# Autodesk Inventor assembly: Clutch Concept
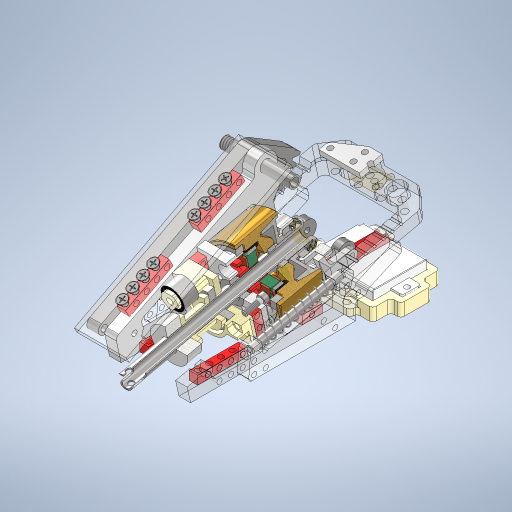
[picture p0: Inventor's stored thumbnail of the model, 512x512]
Saved by Autodesk Inventor 2023.2 (Build 272271000, 271)
## iProperties
Created: 2024-02-03
Part Number: Clutch Concept
Document SubType Name: Assembly
Designer: Nathan Cai
Mass: 1198 g
Surface Area: 3628.58 cm^2
Volume: 470.445 cm^3
Density: 2.54653 g/cm^3
Author: Nathan Cai
## Documents named in this file (50)
- E:\Documents\Inventor\Bleep V1\Clutch Concept.iam
- E:\Documents\Inventor\Bleep V1\Flywheel.ipt
- E:\Documents\Inventor\Bleep V1\Rack.ipt
- E:\Documents\Inventor\Bleep V1\Pin Cap.ipt
- E:\Documents\Inventor\Bleep V1\Thrust Bearing.ipt
- E:\Documents\Inventor\Bleep V1\BB 13x19x4.ipt
- E:\Documents\Inventor\Bleep V1\Cup.ipt
- E:\Documents\Inventor\Bleep V1\1561T741_Stacked Wave Disc Spring\1561T741_Stacked Wave Disc Spring.ipt
- E:\Documents\Inventor\Bleep V1\AKK RS2205 2300KV\AKK RS2205 2300KV.iam
- E:\Documents\Inventor\Bleep V1\Nut Strip 2x1 - 4-40.ipt
- E:\Documents\Inventor\Bleep V1\BB 37mm x 30mm x 4mm.ipt
- E:\Documents\Inventor\Bleep V1\Motor Plate.ipt
- E:\Documents\Inventor\Bleep V1\Uprights.ipt
- E:\Documents\Inventor\Bleep V1\Nut Strip 4x4 - 4-40.ipt
- E:\Documents\Inventor\Bleep V1\5172T23_Metal Gear - 20 Degree Pressure Angle\5172T23_Metal Gear - 20 Degree Pressure Angle.ipt
- E:\Documents\Inventor\Bleep V1\BB .25x.5x.1875 - Flangeless.ipt
- E:\Documents\Inventor\Content Center Files\R2023\en-US\ANSI B18.3(13)\ANSI B18.3 - 4-40 UNC - 0.375(22).ipt
- E:\Documents\Inventor\Bleep V1\Lever.ipt
- E:\Documents\Inventor\Bleep V1\Servo Support.ipt
- E:\Documents\Inventor\Bleep V1\Part1\Part1.ipt
- E:\Documents\Inventor\Bleep V1\Cam - Lever.ipt
- E:\Documents\Inventor\Bleep V1\Cam - Shell.ipt
- E:\Documents\Inventor\Bleep V1\BB 3x7x3.ipt
- E:\Documents\Inventor\Bleep V1\Ramp.ipt
- E:\Documents\Inventor\Content Center Files\R2023\en-US\ANSI B18.6.3(12)\ANSI B18.6.3 - 4-40 UNC - 0.375(15_).ipt
- E:\Documents\Inventor\Content Center Files\R2023\en-US\ISO 4762(2)\ISO 4762 - M3 x 12ISO.ipt
- E:\Documents\Inventor\Content Center Files\R2023\en-US\NF E 25-409\NF E 25-409 - M3.ipt
- E:\Documents\Inventor\Bleep V1\Lever - Copy.ipt
- E:\Documents\Inventor\Bleep V1\Brace.ipt
- E:\Documents\Inventor\Bleep V1\Tattu 4S 850mah\Tattu 850mah 4S.iam
- E:\Documents\Inventor\Bleep V1\BB 3x7x3 - Copy.ipt
- E:\Documents\Inventor\Bleep V1\End Guides - Rail.ipt
- E:\Documents\Inventor\Bleep V1\Spring.ipt
- E:\Documents\Inventor\Bleep V1\Shaft - Arms.ipt
- E:\Documents\Inventor\Bleep V1\Bottom Plate.ipt
- E:\Documents\Inventor\Bleep V1\Side Plate.ipt
- E:\Documents\Inventor\Bleep V1\Top Plate.ipt
- E:\Documents\Inventor\Bleep V1\Back Plate.ipt
- E:\Documents\Inventor\Bleep V1\Uprights- Exterior.ipt
- E:\Documents\Inventor\Bleep V1\Cover.ipt
- E:\Documents\Inventor\Bleep V1\Wheel  - Front.ipt
- E:\Documents\Inventor\Bleep V1\Wheel - Back.ipt
- E:\Documents\Inventor\Bleep V1\Wedge.ipt
- E:\Documents\Inventor\Bleep V1\Ranglebox Mars-25 Assembly - Simple\Ranglebox Mars-25 Assembly - Simple.ipt
- E:\Documents\Inventor\Bleep V1\Shaft - Flywheel C.ipt
- E:\Documents\Inventor\Bleep V1\Clutch C.ipt
- E:\Documents\Inventor\Bleep V1\9293K44_Constant-Force Spring\9293K44_Constant-Force Spring.ipt
- E:\Documents\Inventor\Bleep V1\Spring Mount.ipt
- E:\Documents\Inventor\Bleep V1\Spring Spool.ipt
- E:\Documents\Inventor\Bleep V1\Collar.ipt
## Components (96 placed, 49 different names)
1. 9293K44_Constant-Force Spring:1 — Mate:323, Tangent:2
2. Spring Mount:1 — Mate:316, Flush:149, Mate:317, Mate:320, Mate:323, Tangent:2
3. Thrust Bearing:1 — Mate:319, Mate:320, Mate:322
4. Spring Spool:1 — Mate:321, Mate:322, Mate:325
5. Collar:1 — Mate:324, Mate:325
6. Flywheel:1 — Mate:37, Flush:102, Mate:104, Mate:105, Mate:275, Mate:309
7. Shaft - Flywheel C:1 — Mate:306, Mate:307, Mate:308, Mate:310, Mate:311, Mate:312, Mate:313, Mate:314, Mate:315, Angle:4, Mate:319, Mate:321, Mate:324
8. Shaft - Arms:1 — Mate:257, Flush:118, Mate:288, Mate:291
9. Clutch C:1 — Mate:308, Angle:4
10. Rack:1 — Flush:5, Mate:17, Mate:19, Angle:1, Angle:3, Rotation/Translation:1, Mate:315, Mate:258, Mate:259, Mate:260, Mate:261, Flush:122, Mate:313, Mate:314, Flush:148
11. Pin Cap:1 — Flush:5, Mate:17, Mate:19
12. Cup:1 — Mate:26, Mate:27, Angle:1, Tangent:1
13. 1561T741_Stacked Wave Disc Spring:1 — Mate:311, Mate:312
14. AKK RS2205 2300KV:1 [sub-assembly] — Mate:37, Flush:102, Mate:142
15. Motor Plate:1 — Mate:106, Mate:107, Mate:128, Mate:129, Mate:131, Mate:132, Mate:134, Mate:136, Mate:142, Flush:106, Mate:144, Mate:145, Mate:146, Mate:147, Mate:148, Mate:149, Mate:150, Mate:151, Mate:152, Mate:153, Mate:154, Mate:155, Mate:156, Mate:157, Mate:158, Mate:159, Flush:149
16. Uprights:1 — Mate:128, Mate:130, Flush:103, Flush:104, Mate:133, Mate:138, Mate:141, Flush:107, Mate:168, Mate:169, Flush:108, Mate:229, Mate:230, Flush:110, Mate:257, Mate:265, Mate:266, Mate:267, Mate:268, Mate:269, Flush:125, Mate:317
17. Uprights:2 — Flush:103, Mate:132, Flush:104, Mate:135, Mate:137, Mate:139, Mate:140, Mate:191, Mate:226, Mate:228, Flush:111, Mate:262, Mate:263, Mate:264, Mate:270, Mate:271, Flush:124, Mate:284
18. Brace:1 — Mate:226, Mate:228, Flush:111, Mate:292
19. Brace:2 — Mate:229, Mate:230, Flush:110, Flush:123, Mate:289
20. Nut Strip 4x4 - 4-40:1 — Mate:129, Mate:130, Mate:131, Mate:133, Mate:316
21. Nut Strip 4x4 - 4-40:2 — Mate:134, Mate:135, Mate:136, Mate:137
22. 5172T23_Metal Gear - 20 Degree Pressure Angle:1 — Mate:138, Mate:141, Flush:105, Angle:3, Mate:198, Mate:199, Mate:200, Mate:201, Mate:202, Mate:203, Mate:204, Rotation/Translation:1, Flush:118, Mate:287
23. 5172T23_Metal Gear - 20 Degree Pressure Angle:2 — Mate:139, Mate:140, Flush:105, Mate:192, Mate:193, Mate:194, Mate:195, Mate:196, Mate:197, Mate:290
24. BB .25x.5x.1875 - Flangeless:1 — Flush:106, Mate:310
25. Lever:1 — Mate:168, Mate:169, Tangent:1, Mate:181, Mate:182, Mate:183, Mate:222, Mate:224, Mate:225
26. Lever - Copy:1
27. Part1:1 — Mate:179, Mate:180, Mate:186, Mate:187, Mate:188
28. Cam - Lever:1 — Mate:177, Mate:178, Mate:183
29. Cam - Shell:1 — Mate:177, Mate:178, Mate:179, Mate:180
30. BB 3x7x3:1 — Mate:181, Mate:182
31. BB 3x7x3:2
32. BB 3x7x3 - Copy:1
33. BB 13x19x4:1 — Mate:26, Mate:27
34. BB 37mm x 30mm x 4mm:1 — Mate:104, Mate:105, Mate:106, Mate:107
35. BB .25x.5x.1875 - Flangeless:2 — Mate:275, Mate:306, Mate:307, Mate:309
36. Servo Support:1 — Mate:186, Mate:187, Mate:188, Flush:108, Mate:191, Flush:136
37. Ramp:1 — Mate:204, Mate:205, Mate:206, Mate:207, Mate:208, Mate:209, Mate:210, Mate:211, Mate:212, Mate:213, Mate:214, Mate:215, Mate:216, Mate:217, Mate:218, Mate:219, Mate:220, Mate:221, Mate:304
38. Nut Strip 4x4 - 4-40:3 — Mate:192, Mate:193, Mate:194, Mate:304
39. Nut Strip 4x4 - 4-40:5 — Mate:199, Mate:200, Mate:201
40. Nut Strip 4x4 - 4-40:6 — Mate:198, Mate:202, Mate:203, Mate:205
41. Nut Strip 4x4 - 4-40:7 — Mate:195, Mate:196, Mate:197
42. Nut Strip 4x4 - 4-40:8 — Mate:265, Mate:266, Mate:267
43. Nut Strip 4x4 - 4-40:9 — Mate:262, Mate:263, Mate:264
44. Nut Strip 2x1 - 4-40:3 — Mate:270, Mate:271, Flush:124
45. Nut Strip 2x1 - 4-40:4 — Mate:268, Mate:269, Flush:125
46. End Guides - Rail:1 — Mate:243, Mate:258, Mate:259
47. End Guides - Rail:2 — Mate:260, Mate:261
48. Spring:1 — Mate:243, Flush:122, Flush:123
49. Spring:2 — Flush:148
50. Cross Recessed Flat Countersunk Head Machine Screw - Type I - Inch 4-40 x 3/8:1 — Mate:206
51. Cross Recessed Flat Countersunk Head Machine Screw - Type I - Inch 4-40 x 3/8:2 — Mate:207
52. Cross Recessed Flat Countersunk Head Machine Screw - Type I - Inch 4-40 x 3/8:3 — Mate:208
53. Cross Recessed Flat Countersunk Head Machine Screw - Type I - Inch 4-40 x 3/8:4 — Mate:209
54. Cross Recessed Flat Countersunk Head Machine Screw - Type I - Inch 4-40 x 3/8:5 — Mate:210
55. Cross Recessed Flat Countersunk Head Machine Screw - Type I - Inch 4-40 x 3/8:6 — Mate:211
56. Cross Recessed Flat Countersunk Head Machine Screw - Type I - Inch 4-40 x 3/8:7 — Mate:212
57. Cross Recessed Flat Countersunk Head Machine Screw - Type I - Inch 4-40 x 3/8:8 — Mate:213
58. Cross Recessed Flat Countersunk Head Machine Screw - Type I - Inch 4-40 x 3/8:9 — Mate:214
59. Cross Recessed Flat Countersunk Head Machine Screw - Type I - Inch 4-40 x 3/8:10 — Mate:215
60. Cross Recessed Flat Countersunk Head Machine Screw - Type I - Inch 4-40 x 3/8:11 — Mate:216
61. Cross Recessed Flat Countersunk Head Machine Screw - Type I - Inch 4-40 x 3/8:12 — Mate:217
62. Cross Recessed Flat Countersunk Head Machine Screw - Type I - Inch 4-40 x 3/8:13 — Mate:218
63. Cross Recessed Flat Countersunk Head Machine Screw - Type I - Inch 4-40 x 3/8:14 — Mate:219
64. Cross Recessed Flat Countersunk Head Machine Screw - Type I - Inch 4-40 x 3/8:15 — Mate:220
65. Cross Recessed Flat Countersunk Head Machine Screw - Type I - Inch 4-40 x 3/8:16 — Mate:221
66. ISO 4762 M3 x 12:1 — Mate:222
67. NF E 25-409 M3:1 — Mate:224, Mate:225
68. Spline Socket Head Cap Screw - Inch 4-40 UNC - 0.375:1 — Mate:144, Mate:145
69. Spline Socket Head Cap Screw - Inch 4-40 UNC - 0.375:2 — Mate:146, Mate:147
70. Spline Socket Head Cap Screw - Inch 4-40 UNC - 0.375:3 — Mate:148, Mate:149
71. Spline Socket Head Cap Screw - Inch 4-40 UNC - 0.375:4 — Mate:150, Mate:151
72. Spline Socket Head Cap Screw - Inch 4-40 UNC - 0.375:5 — Mate:152, Mate:153
73. Spline Socket Head Cap Screw - Inch 4-40 UNC - 0.375:6 — Mate:154, Mate:155
74. Spline Socket Head Cap Screw - Inch 4-40 UNC - 0.375:7 — Mate:156, Mate:157
75. Spline Socket Head Cap Screw - Inch 4-40 UNC - 0.375:8 — Mate:158, Mate:159
76. Tattu 850mah 4S:1 [sub-assembly]
77. Bottom Plate:1 — Mate:278, Flush:127, Flush:128, Mate:279, Flush:129, Flush:130, Flush:131, Flush:136, Mate:284, Mate:285, Flush:143
78. Side Plate:1 — Mate:278, Flush:127, Flush:128, Mate:280, Flush:134, Flush:135, Mate:282, Flush:140, Flush:141, Mate:286, Flush:147
79. Side Plate:2 — Mate:279, Flush:129, Flush:130, Mate:281, Flush:137, Flush:138, Mate:283, Flush:139, Flush:142, Flush:146
80. Top Plate:1 — Mate:280, Flush:134, Flush:135
81. Top Plate:2 — Mate:281, Flush:137, Flush:138
82. Side Plate:3 — Mate:282, Flush:140, Flush:141
83. Side Plate:4 — Mate:283, Flush:139, Flush:142
84. Back Plate:1 — Mate:285, Flush:143, Mate:286
85. Uprights- Exterior:1 — Mate:287, Mate:288, Mate:289, Mate:293, Mate:294, Mate:295, Flush:144
86. Uprights- Exterior:2 — Mate:290, Mate:291, Mate:292, Mate:296, Mate:297, Mate:298
87. Nut Strip 4x4 - 4-40:10 — Mate:293, Mate:294, Mate:295
88. Nut Strip 4x4 - 4-40:11 — Mate:296, Mate:297, Mate:298, Mate:299
89. Cover:1 — Mate:299, Flush:144
90. Wheel  - Front:1 — Flush:145, Mate:302
91. Wheel - Back:1 — Flush:145, Mate:301
92. Wheel  - Front:2 — Mate:302
93. Wheel - Back:2 — Mate:301
94. Wedge:1
95. Ranglebox Mars-25 Assembly - Simple:1 — Mate:303, Flush:146
96. Ranglebox Mars-25 Assembly - Simple:2 — Mate:303, Flush:147
## Relationships (205: Mate 163, Flush 36, Angle 3, Tangent 2, RelateRotateTranslate 1)
- Flush:5: Rack:1 ↔ Pin Cap:1
- Mate:17: Rack:1 ↔ Pin Cap:1
- Mate:19: Rack:1 ↔ Pin Cap:1
- [Mate]: Clutch C:1 ↔ BB 13x19x4:1
- [Mate]: Clutch C:1 ↔ BB 13x19x4:1
- Mate:26: Cup:1 ↔ BB 13x19x4:1
- Mate:27: Cup:1 ↔ BB 13x19x4:1
- Mate:37: Flywheel:1 ↔ AKK RS2205 2300KV:1
- Angle:1 (0 deg): Rack:1 ↔ Cup:1
- Flush:102: Flywheel:1 ↔ AKK RS2205 2300KV:1
- Mate:104: Flywheel:1 ↔ BB 37mm x 30mm x 4mm:1
- Mate:105: Flywheel:1 ↔ BB 37mm x 30mm x 4mm:1
- Mate:106: Motor Plate:1 ↔ BB 37mm x 30mm x 4mm:1
- Mate:107: Motor Plate:1 ↔ BB 37mm x 30mm x 4mm:1
- Mate:128: Motor Plate:1 ↔ Uprights:1
- Mate:129: Motor Plate:1 ↔ Nut Strip 4x4 - 4-40:1
- Mate:130: Uprights:1 ↔ Nut Strip 4x4 - 4-40:1
- Mate:131: Motor Plate:1 ↔ Nut Strip 4x4 - 4-40:1
- Flush:103: Uprights:1 ↔ Uprights:2
- Mate:132: Motor Plate:1 ↔ Uprights:2
- Flush:104: Uprights:1 ↔ Uprights:2
- Mate:133: Uprights:1 ↔ Nut Strip 4x4 - 4-40:1
- Mate:134: Motor Plate:1 ↔ Nut Strip 4x4 - 4-40:2
- Mate:135: Uprights:2 ↔ Nut Strip 4x4 - 4-40:2
- Mate:136: Motor Plate:1 ↔ Nut Strip 4x4 - 4-40:2
- Mate:137: Uprights:2 ↔ Nut Strip 4x4 - 4-40:2
- Mate:138: Uprights:1 ↔ 5172T23_Metal Gear - 20 Degree Pressure Angle:1
- Mate:139: Uprights:2 ↔ 5172T23_Metal Gear - 20 Degree Pressure Angle:2
- Mate:140: Uprights:2 ↔ 5172T23_Metal Gear - 20 Degree Pressure Angle:2
- Mate:141: Uprights:1 ↔ 5172T23_Metal Gear - 20 Degree Pressure Angle:1
- Flush:105: 5172T23_Metal Gear - 20 Degree Pressure Angle:1 ↔ 5172T23_Metal Gear - 20 Degree Pressure Angle:2
- Mate:142: AKK RS2205 2300KV:1 ↔ Motor Plate:1
- Flush:106: Motor Plate:1 ↔ BB .25x.5x.1875 - Flangeless:1
- Mate:144: Motor Plate:1 ↔ Spline Socket Head Cap Screw - Inch 4-40 UNC - 0.375:1
- Mate:145: Motor Plate:1 ↔ Spline Socket Head Cap Screw - Inch 4-40 UNC - 0.375:1
- Mate:146: Motor Plate:1 ↔ Spline Socket Head Cap Screw - Inch 4-40 UNC - 0.375:2
- Mate:147: Motor Plate:1 ↔ Spline Socket Head Cap Screw - Inch 4-40 UNC - 0.375:2
- Mate:148: Motor Plate:1 ↔ Spline Socket Head Cap Screw - Inch 4-40 UNC - 0.375:3
- Mate:149: Motor Plate:1 ↔ Spline Socket Head Cap Screw - Inch 4-40 UNC - 0.375:3
- Mate:150: Motor Plate:1 ↔ Spline Socket Head Cap Screw - Inch 4-40 UNC - 0.375:4
- Mate:151: Motor Plate:1 ↔ Spline Socket Head Cap Screw - Inch 4-40 UNC - 0.375:4
- Mate:152: Motor Plate:1 ↔ Spline Socket Head Cap Screw - Inch 4-40 UNC - 0.375:5
- Mate:153: Motor Plate:1 ↔ Spline Socket Head Cap Screw - Inch 4-40 UNC - 0.375:5
- Mate:154: Motor Plate:1 ↔ Spline Socket Head Cap Screw - Inch 4-40 UNC - 0.375:6
- Mate:155: Motor Plate:1 ↔ Spline Socket Head Cap Screw - Inch 4-40 UNC - 0.375:6
- Mate:156: Motor Plate:1 ↔ Spline Socket Head Cap Screw - Inch 4-40 UNC - 0.375:7
- Mate:157: Motor Plate:1 ↔ Spline Socket Head Cap Screw - Inch 4-40 UNC - 0.375:7
- Mate:158: Motor Plate:1 ↔ Spline Socket Head Cap Screw - Inch 4-40 UNC - 0.375:8
- Mate:159: Motor Plate:1 ↔ Spline Socket Head Cap Screw - Inch 4-40 UNC - 0.375:8
- Flush:107: Uprights:1
- Mate:168: Uprights:1 ↔ Lever:1
- Mate:169: Uprights:1 ↔ Lever:1
- Tangent:1: Cup:1 ↔ Lever:1
- Angle:3 (0 deg): Rack:1 ↔ 5172T23_Metal Gear - 20 Degree Pressure Angle:1
- [Mate]: Uprights:2 ↔ Lever - Copy:1
- [Mate]: Uprights:2 ↔ Lever - Copy:1
- [Mate]: Lever:1 ↔ Lever - Copy:1
- Mate:177: Cam - Lever:1 ↔ Cam - Shell:1
- Mate:178: Cam - Lever:1 ↔ Cam - Shell:1
- Mate:179: Part1:1 ↔ Cam - Shell:1
- Mate:180: Part1:1 ↔ Cam - Shell:1
- Mate:181: Lever:1 ↔ BB 3x7x3:1
- Mate:182: Lever:1 ↔ BB 3x7x3:1
- Mate:183: Lever:1 ↔ Cam - Lever:1
- [Mate]: Lever - Copy:1 ↔ BB 3x7x3:2
- [Mate]: Lever - Copy:1 ↔ BB 3x7x3:2
- Mate:186: Part1:1 ↔ Servo Support:1
- Mate:187: Part1:1 ↔ Servo Support:1
- Mate:188: Part1:1 ↔ Servo Support:1
- Flush:108: Uprights:1 ↔ Servo Support:1
- [Mate]: Lever:1 ↔ BB 3x7x3 - Copy:1
- [Mate]: Lever:1 ↔ BB 3x7x3 - Copy:1
- Mate:191: Uprights:2 ↔ Servo Support:1
- Mate:192: 5172T23_Metal Gear - 20 Degree Pressure Angle:2 ↔ Nut Strip 4x4 - 4-40:3
- Mate:193: 5172T23_Metal Gear - 20 Degree Pressure Angle:2 ↔ Nut Strip 4x4 - 4-40:3
- Mate:194: 5172T23_Metal Gear - 20 Degree Pressure Angle:2 ↔ Nut Strip 4x4 - 4-40:3
- Mate:195: 5172T23_Metal Gear - 20 Degree Pressure Angle:2 ↔ Nut Strip 4x4 - 4-40:7
- Mate:196: 5172T23_Metal Gear - 20 Degree Pressure Angle:2 ↔ Nut Strip 4x4 - 4-40:7
- Mate:197: 5172T23_Metal Gear - 20 Degree Pressure Angle:2 ↔ Nut Strip 4x4 - 4-40:7
- Mate:198: 5172T23_Metal Gear - 20 Degree Pressure Angle:1 ↔ Nut Strip 4x4 - 4-40:6
- Mate:199: 5172T23_Metal Gear - 20 Degree Pressure Angle:1 ↔ Nut Strip 4x4 - 4-40:5
- Mate:200: 5172T23_Metal Gear - 20 Degree Pressure Angle:1 ↔ Nut Strip 4x4 - 4-40:5
- Mate:201: 5172T23_Metal Gear - 20 Degree Pressure Angle:1 ↔ Nut Strip 4x4 - 4-40:5
- Mate:202: 5172T23_Metal Gear - 20 Degree Pressure Angle:1 ↔ Nut Strip 4x4 - 4-40:6
- Mate:203: 5172T23_Metal Gear - 20 Degree Pressure Angle:1 ↔ Nut Strip 4x4 - 4-40:6
- Mate:204: 5172T23_Metal Gear - 20 Degree Pressure Angle:1 ↔ Ramp:1
- Mate:205: Ramp:1 ↔ Nut Strip 4x4 - 4-40:6
- Mate:206: Ramp:1 ↔ Cross Recessed Flat Countersunk Head Machine Screw - Type I - Inch 4-40 x 3/8:1
- Mate:207: Ramp:1 ↔ Cross Recessed Flat Countersunk Head Machine Screw - Type I - Inch 4-40 x 3/8:2
- Mate:208: Ramp:1 ↔ Cross Recessed Flat Countersunk Head Machine Screw - Type I - Inch 4-40 x 3/8:3
- Mate:209: Ramp:1 ↔ Cross Recessed Flat Countersunk Head Machine Screw - Type I - Inch 4-40 x 3/8:4
- Mate:210: Ramp:1 ↔ Cross Recessed Flat Countersunk Head Machine Screw - Type I - Inch 4-40 x 3/8:5
- Mate:211: Ramp:1 ↔ Cross Recessed Flat Countersunk Head Machine Screw - Type I - Inch 4-40 x 3/8:6
- Mate:212: Ramp:1 ↔ Cross Recessed Flat Countersunk Head Machine Screw - Type I - Inch 4-40 x 3/8:7
- Mate:213: Ramp:1 ↔ Cross Recessed Flat Countersunk Head Machine Screw - Type I - Inch 4-40 x 3/8:8
- Mate:214: Ramp:1 ↔ Cross Recessed Flat Countersunk Head Machine Screw - Type I - Inch 4-40 x 3/8:9
- Mate:215: Ramp:1 ↔ Cross Recessed Flat Countersunk Head Machine Screw - Type I - Inch 4-40 x 3/8:10
- Mate:216: Ramp:1 ↔ Cross Recessed Flat Countersunk Head Machine Screw - Type I - Inch 4-40 x 3/8:11
- Mate:217: Ramp:1 ↔ Cross Recessed Flat Countersunk Head Machine Screw - Type I - Inch 4-40 x 3/8:12
- Mate:218: Ramp:1 ↔ Cross Recessed Flat Countersunk Head Machine Screw - Type I - Inch 4-40 x 3/8:13
- Mate:219: Ramp:1 ↔ Cross Recessed Flat Countersunk Head Machine Screw - Type I - Inch 4-40 x 3/8:14
- Mate:220: Ramp:1 ↔ Cross Recessed Flat Countersunk Head Machine Screw - Type I - Inch 4-40 x 3/8:15
- Mate:221: Ramp:1 ↔ Cross Recessed Flat Countersunk Head Machine Screw - Type I - Inch 4-40 x 3/8:16
- Mate:222: Lever:1 ↔ ISO 4762 M3 x 12:1
- [Mate]: BB 3x7x3 - Copy:1 ↔ ISO 4762 M3 x 12:1
- Mate:224: Lever:1 ↔ NF E 25-409 M3:1
- Mate:225: Lever:1 ↔ NF E 25-409 M3:1
- Mate:226: Uprights:2 ↔ Brace:1
- Mate:228: Uprights:2 ↔ Brace:1
- Mate:229: Uprights:1 ↔ Brace:2
- Mate:230: Uprights:1 ↔ Brace:2
- Rotation/Translation:1 [RelateRotateTranslate] (159.5929 mm): Rack:1 ↔ 5172T23_Metal Gear - 20 Degree Pressure Angle:1
- Flush:110: Uprights:1 ↔ Brace:2
- Flush:111: Uprights:2 ↔ Brace:1
- Mate:243: End Guides - Rail:1 ↔ Spring:1
- [Mate]: End Guides - Rail:2 ↔ Spring:2
- Mate:257: Shaft - Arms:1 ↔ Uprights:1
- Flush:118 (-9.525 mm): Shaft - Arms:1 ↔ 5172T23_Metal Gear - 20 Degree Pressure Angle:1
- Mate:315 (31.75 mm): Shaft - Flywheel C:1 ↔ Rack:1
- Mate:258 (0.7937 mm): Rack:1 ↔ End Guides - Rail:1
- Mate:259: Rack:1 ↔ End Guides - Rail:1
- Mate:260 (0.7937 mm): Rack:1 ↔ End Guides - Rail:2
- Mate:261: Rack:1 ↔ End Guides - Rail:2
- Flush:122: Rack:1 ↔ Spring:1
- Flush:123: Brace:2 ↔ Spring:1
- Mate:262: Uprights:2 ↔ Nut Strip 4x4 - 4-40:9
- Mate:263: Uprights:2 ↔ Nut Strip 4x4 - 4-40:9
- Mate:264: Uprights:2 ↔ Nut Strip 4x4 - 4-40:9
- Mate:265: Uprights:1 ↔ Nut Strip 4x4 - 4-40:8
- Mate:266: Uprights:1 ↔ Nut Strip 4x4 - 4-40:8
- Mate:267: Uprights:1 ↔ Nut Strip 4x4 - 4-40:8
- Mate:268: Uprights:1 ↔ Nut Strip 2x1 - 4-40:4
- Mate:269: Uprights:1 ↔ Nut Strip 2x1 - 4-40:4
- Mate:270: Uprights:2 ↔ Nut Strip 2x1 - 4-40:3
- Mate:271: Uprights:2 ↔ Nut Strip 2x1 - 4-40:3
- Flush:124: Uprights:2 ↔ Nut Strip 2x1 - 4-40:3
- Flush:125: Uprights:1 ↔ Nut Strip 2x1 - 4-40:4
- Mate:275: Flywheel:1 ↔ BB .25x.5x.1875 - Flangeless:2
- Mate:278: Bottom Plate:1 ↔ Side Plate:1
- Flush:127: Bottom Plate:1 ↔ Side Plate:1
- Flush:128: Bottom Plate:1 ↔ Side Plate:1
- Mate:279: Bottom Plate:1 ↔ Side Plate:2
- Flush:129: Bottom Plate:1 ↔ Side Plate:2
- Flush:130: Bottom Plate:1 ↔ Side Plate:2
- Flush:131: Bottom Plate:1
- Mate:280: Side Plate:1 ↔ Top Plate:1
- Flush:134: Side Plate:1 ↔ Top Plate:1
- Flush:135: Side Plate:1 ↔ Top Plate:1
- Flush:136 (9.525 mm): Servo Support:1 ↔ Bottom Plate:1
- Mate:281: Side Plate:2 ↔ Top Plate:2
- Flush:137: Side Plate:2 ↔ Top Plate:2
- Flush:138: Side Plate:2 ↔ Top Plate:2
- Mate:282 (25.4 mm): Side Plate:1 ↔ Side Plate:3
- Mate:283 (25.4 mm): Side Plate:2 ↔ Side Plate:4
- Flush:139: Side Plate:2 ↔ Side Plate:4
- Flush:140: Side Plate:1 ↔ Side Plate:3
- Flush:141: Side Plate:1 ↔ Side Plate:3
- Flush:142: Side Plate:2 ↔ Side Plate:4
- Mate:284: Uprights:2 ↔ Bottom Plate:1
- Mate:285: Bottom Plate:1 ↔ Back Plate:1
- Flush:143: Bottom Plate:1 ↔ Back Plate:1
- Mate:286: Side Plate:1 ↔ Back Plate:1
- Mate:287: 5172T23_Metal Gear - 20 Degree Pressure Angle:1 ↔ Uprights- Exterior:1
- Mate:288: Shaft - Arms:1 ↔ Uprights- Exterior:1
- Mate:289: Brace:2 ↔ Uprights- Exterior:1
- Mate:290: 5172T23_Metal Gear - 20 Degree Pressure Angle:2 ↔ Uprights- Exterior:2
- Mate:291: Shaft - Arms:1 ↔ Uprights- Exterior:2
- Mate:292: Brace:1 ↔ Uprights- Exterior:2
- Mate:293: Uprights- Exterior:1 ↔ Nut Strip 4x4 - 4-40:10
- Mate:294: Uprights- Exterior:1 ↔ Nut Strip 4x4 - 4-40:10
- Mate:295: Uprights- Exterior:1 ↔ Nut Strip 4x4 - 4-40:10
- Mate:296: Uprights- Exterior:2 ↔ Nut Strip 4x4 - 4-40:11
- Mate:297: Uprights- Exterior:2 ↔ Nut Strip 4x4 - 4-40:11
- Mate:298: Uprights- Exterior:2 ↔ Nut Strip 4x4 - 4-40:11
- Mate:299: Nut Strip 4x4 - 4-40:11 ↔ Cover:1
- Flush:144: Uprights- Exterior:1 ↔ Cover:1
- Flush:145: Wheel  - Front:1 ↔ Wheel - Back:1
- Mate:301: Wheel - Back:1 ↔ Wheel - Back:2
- Mate:302: Wheel  - Front:1 ↔ Wheel  - Front:2
- Mate:303: Ranglebox Mars-25 Assembly - Simple:1 ↔ Ranglebox Mars-25 Assembly - Simple:2
- Flush:146: Side Plate:2 ↔ Ranglebox Mars-25 Assembly - Simple:1
- Flush:147: Side Plate:1 ↔ Ranglebox Mars-25 Assembly - Simple:2
- Mate:304: Ramp:1 ↔ Nut Strip 4x4 - 4-40:3
- Mate:306: Shaft - Flywheel C:1 ↔ BB .25x.5x.1875 - Flangeless:2
- Mate:307: Shaft - Flywheel C:1 ↔ BB .25x.5x.1875 - Flangeless:2
- Mate:308: Shaft - Flywheel C:1 ↔ Clutch C:1
- Mate:309: Flywheel:1 ↔ BB .25x.5x.1875 - Flangeless:2
- Mate:310: Shaft - Flywheel C:1 ↔ BB .25x.5x.1875 - Flangeless:1
- Mate:311: Shaft - Flywheel C:1 ↔ 1561T741_Stacked Wave Disc Spring:1
- Mate:312: Shaft - Flywheel C:1 ↔ 1561T741_Stacked Wave Disc Spring:1
- Mate:313: Shaft - Flywheel C:1 ↔ Rack:1
- Mate:314: Shaft - Flywheel C:1 ↔ Rack:1
- Flush:148: Rack:1 ↔ Spring:2
- Angle:4 (0 deg): Shaft - Flywheel C:1 ↔ Clutch C:1
- Mate:316: Spring Mount:1 ↔ Nut Strip 4x4 - 4-40:1
- Flush:149 (2.3813 mm): Spring Mount:1 ↔ Motor Plate:1
- Mate:317: Spring Mount:1 ↔ Uprights:1
- Mate:319: Thrust Bearing:1 ↔ Shaft - Flywheel C:1
- Mate:320: Spring Mount:1 ↔ Thrust Bearing:1
- Mate:321: Spring Spool:1 ↔ Shaft - Flywheel C:1
- Mate:322: Thrust Bearing:1 ↔ Spring Spool:1
- Mate:323: 9293K44_Constant-Force Spring:1 ↔ Spring Mount:1
- Mate:324: Collar:1 ↔ Shaft - Flywheel C:1
- Mate:325: Spring Spool:1 ↔ Collar:1
- Tangent:2: 9293K44_Constant-Force Spring:1 ↔ Spring Mount:1
## Named parameters: d530_d520 = 0 mm
